# Autodesk Inventor assembly: castor_assembly
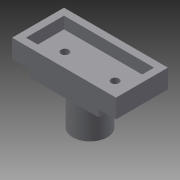
[picture p0: Inventor's stored thumbnail of the model, 180x180]
Saved by Autodesk Inventor 2015 (Build 190159000, 159)
## iProperties
Created: 2014-11-12
Part Number: castor_assembly
Document SubType Name: Assembly
Designer: Colin
Author: Colin
## Documents named in this file (3)
- E:\Users\Colin\Documents\college\marc\MicroMouse\castor_assembly.iam
- E:\Users\Colin\Documents\college\marc\MicroMouse\castor_bracket.ipt
- E:\Users\Colin\Documents\college\marc\MicroMouse\half_inch_castor.ipt
## Components (2 placed, 2 different names)
1. castor_bracket:1 — Mate:1, Mate:2, Mate:3
2. half_inch_castor:1 — Mate:1, Mate:2, Mate:3
## Relationships (3: Mate 3)
- Mate:1: castor_bracket:1 ↔ half_inch_castor:1
- Mate:2: castor_bracket:1 ↔ half_inch_castor:1
- Mate:3: castor_bracket:1 ↔ half_inch_castor:1
